# Autodesk Inventor assembly: ASS_Roue_Libre
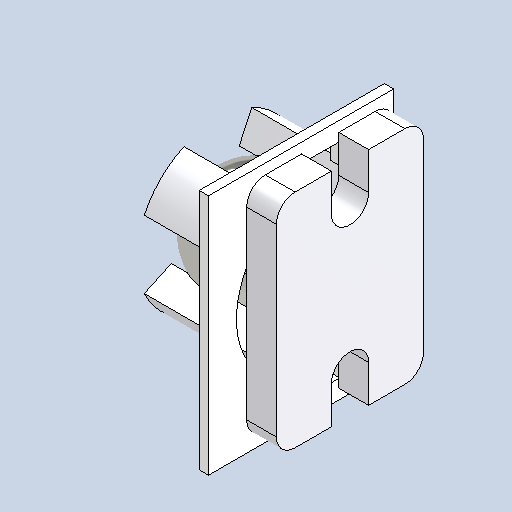
[picture p0: Inventor's stored thumbnail of the model, 512x512]
Saved by Autodesk Inventor 2022 (Build 260153000, 153)
## iProperties
Created: 2022-03-23
Part Number: ASS_Roue_Libre
Document SubType Name: Assembly
Designer: utilisateur
Author: utilisateur
## Documents named in this file (3)
- C:\Users\victo\Desktop\Documents\ENSTA\Cours ENSTA\2A\PIE\Modélisation\Robot réduit\ASS_Roue_Libre-20220506T114758Z-001\ASS_Roue_Libre\ASS_Roue_Libre.iam
- C:\Users\victo\Desktop\Documents\ENSTA\Cours ENSTA\2A\PIE\Modélisation\Robot réduit\ASS_Roue_Libre-20220506T114758Z-001\ASS_Roue_Libre\Roue_libre.ipt
- C:\Users\victo\Desktop\Documents\ENSTA\Cours ENSTA\2A\PIE\Modélisation\Robot réduit\ASS_Roue_Libre-20220506T114758Z-001\ASS_Roue_Libre\Fi_Roue_Libre_P.ipt
## Components (2 placed, 2 different names)
1. Roue_libre:1 — Mate:1, Mate:2, Mate:3, Mate:6, Mate:7
2. Fi_Roue_Libre_P:1 — Mate:5, Mate:6, Mate:7
## Relationships (6: Mate 6)
- Mate:1: Roue_libre:1
- Mate:2: Roue_libre:1
- Mate:3: Roue_libre:1
- Mate:5: Fi_Roue_Libre_P:1
- Mate:6: Roue_libre:1 ↔ Fi_Roue_Libre_P:1
- Mate:7: Roue_libre:1 ↔ Fi_Roue_Libre_P:1
